# Autodesk Inventor assembly: Head Cylinder and Frame Subassembly
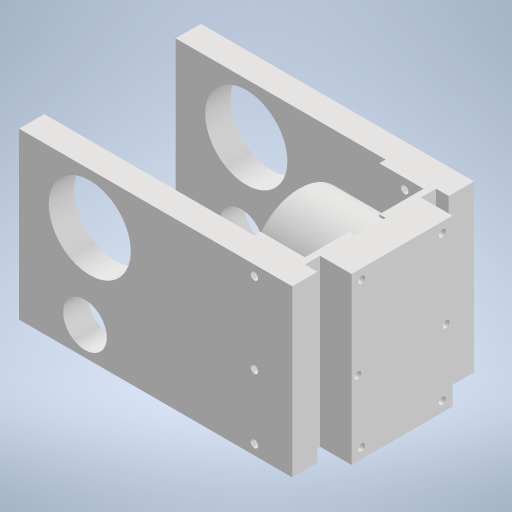
[picture p0: Inventor's stored thumbnail of the model, 512x512]
Saved by Autodesk Inventor 2023 (Build 270158000, 158)
## iProperties
Created: 2022-12-23
Part Number: Head Cylinder and Frame Subassembly
Document SubType Name: Assembly
Designer: tgr41
Author: tgr41
## Documents named in this file (7)
- C:\Users\tgr41\OneDrive\Documents\Repositories\Steam-Engine\2 Inch V3\Head Cylinder and Frame Subassembly.iam
- C:\Users\tgr41\OneDrive\Documents\Repositories\Steam-Engine\2 Inch V3\Engine Head Bottom.ipt
- C:\Users\tgr41\OneDrive\Documents\Repositories\Steam-Engine\2 Inch V3\Engine Head Gasket.ipt
- C:\Users\tgr41\OneDrive\Documents\Repositories\Steam-Engine\2 Inch V3\Engine Head Top.ipt
- C:\Users\tgr41\OneDrive\Documents\Repositories\Steam-Engine\2 Inch V3\Frame L Branket.ipt
- C:\Users\tgr41\OneDrive\Documents\Repositories\Steam-Engine\2 Inch V3\Frame L Branket Opposite Side.ipt
- C:\Users\tgr41\OneDrive\Documents\Repositories\Steam-Engine\2 Inch V3\Frame Sides.ipt
## Components (7 placed, 6 different names)
1. Engine Head Bottom:1 — Mate:1, Mate:2, Mate:3, Mate:7, Mate:8, Mate:9, Mate:10, Mate:11, Mate:12
2. Engine Head Gasket:1 — Mate:1, Mate:2, Mate:3, Mate:4, Mate:5, Mate:6
3. Engine Head Top:1 — Mate:4, Mate:5, Mate:6
4. Frame L Branket:1 — Mate:8, Mate:11, Mate:12, Mate:13, Mate:17, Mate:18
5. Frame L Branket Opposite Side:1 — Mate:7, Mate:9, Mate:10, Mate:14, Mate:15, Mate:16
6. Frame Sides:1 — Mate:13, Mate:17, Mate:18
7. Frame Sides:2 — Mate:14, Mate:15, Mate:16
## Relationships (18: Mate 18)
- Mate:1: Engine Head Bottom:1 ↔ Engine Head Gasket:1
- Mate:2: Engine Head Bottom:1 ↔ Engine Head Gasket:1
- Mate:3: Engine Head Bottom:1 ↔ Engine Head Gasket:1
- Mate:4: Engine Head Gasket:1 ↔ Engine Head Top:1
- Mate:5: Engine Head Gasket:1 ↔ Engine Head Top:1
- Mate:6: Engine Head Gasket:1 ↔ Engine Head Top:1
- Mate:7: Engine Head Bottom:1 ↔ Frame L Branket Opposite Side:1
- Mate:8: Engine Head Bottom:1 ↔ Frame L Branket:1
- Mate:9: Engine Head Bottom:1 ↔ Frame L Branket Opposite Side:1
- Mate:10: Engine Head Bottom:1 ↔ Frame L Branket Opposite Side:1
- Mate:11: Engine Head Bottom:1 ↔ Frame L Branket:1
- Mate:12: Engine Head Bottom:1 ↔ Frame L Branket:1
- Mate:13: Frame L Branket:1 ↔ Frame Sides:1
- Mate:14: Frame L Branket Opposite Side:1 ↔ Frame Sides:2
- Mate:15: Frame L Branket Opposite Side:1 ↔ Frame Sides:2
- Mate:16: Frame L Branket Opposite Side:1 ↔ Frame Sides:2
- Mate:17: Frame L Branket:1 ↔ Frame Sides:1
- Mate:18: Frame L Branket:1 ↔ Frame Sides:1
